# Autodesk Inventor assembly: ForeArmAssembly
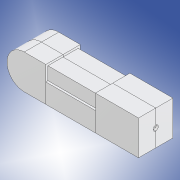
[picture p0: Inventor's stored thumbnail of the model, 180x180]
Saved by Autodesk Inventor 2017 SP1 (Build 210196100, 196)
## iProperties
Created: 2017-06-16
Part Number: ForeArmAssembly
Document SubType Name: Assembly
Designer: Zach
Author: Zach
## Documents named in this file (6)
- C:\Users\Zach\Documents\GitHub\cr-laundry-robot\src\Body\Arm Assembly\Fore Arm Assembly\ForeArmAssembly.iam
- C:\Users\Zach\Documents\GitHub\cr-laundry-robot\src\Body\Arm Assembly\Fore Arm Assembly\FA001.ipt
- C:\Users\Zach\Documents\GitHub\cr-laundry-robot\src\Body\Arm Assembly\Fore Arm Assembly\FA002.ipt
- C:\Users\Zach\Documents\GitHub\cr-laundry-robot\src\Body\Arm Assembly\Fore Arm Assembly\FA003.ipt
- C:\Users\Zach\Documents\GitHub\cr-laundry-robot\src\Body\Arm Assembly\Fore Arm Assembly\FA004.ipt
- C:\Users\Zach\Documents\GitHub\cr-laundry-robot\src\Body\Arm Assembly\Fore Arm Assembly\FA005.ipt
## Components (6 placed, 5 different names)
1. FA001:1 — Mate:1, Mate:2, Mate:3, Mate:4
2. FA002:1 — Mate:1, Mate:2, Mate:5, Mate:6
3. FA003:1 — Mate:3, Mate:4, Mate:10, Mate:11
4. FA003:2 — Mate:5, Mate:6, Mate:8, Mate:9
5. FA004:1 — Mate:8, Mate:9
6. FA005:1 — Mate:10, Mate:11
## Relationships (10: Mate 10)
- Mate:1: FA001:1 ↔ FA002:1
- Mate:2: FA001:1 ↔ FA002:1
- Mate:3: FA001:1 ↔ FA003:1
- Mate:4: FA001:1 ↔ FA003:1
- Mate:5: FA002:1 ↔ FA003:2
- Mate:6: FA002:1 ↔ FA003:2
- Mate:8: FA003:2 ↔ FA004:1
- Mate:9: FA003:2 ↔ FA004:1
- Mate:10: FA003:1 ↔ FA005:1
- Mate:11: FA003:1 ↔ FA005:1
